# Autodesk Inventor assembly: Monitor
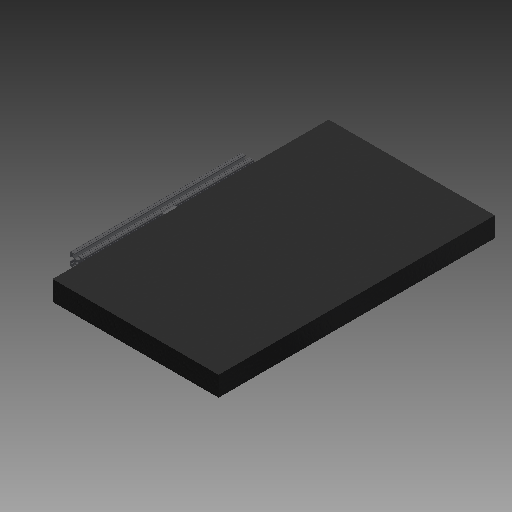
[picture p0: Inventor's stored thumbnail of the model, 512x512]
Saved by Autodesk Inventor 2017 SP1 (Build 210196100, 196)
## iProperties
Created: 2016-04-03
Part Number: Monitor
Document SubType Name: Assembly
Designer: hwasserb
Author: hwasserb
## Documents named in this file (7)
- C:\Users\Haden\Desktop\Charlie-CAD-Model\Robot Model\Monitor\Monitor.iam
- C:\Users\Haden\Desktop\Charlie-CAD-Model\Robot Model\Monitor\Cross Bar.ipt
- C:\Users\Haden\Desktop\Charlie-CAD-Model\Robot Model\Monitor\Monitor.ipt
- C:\Users\Haden\Desktop\Charlie-CAD-Model\Robot Model\Monitor\Vertical Bar.ipt
- C:\Users\Haden\Desktop\Charlie-CAD-Model\Robot Model\Monitor\Lower VESA Mount.ipt
- C:\Users\Haden\Desktop\Charlie-CAD-Model\Robot Model\Monitor\Upper VESA Mount.ipt
- C:\Users\Haden\Desktop\Charlie-CAD-Model\Robot Model\Monitor\Structural Pivot-8020-4198\Structural Pivot-8020-4198.iam
## Components (7 placed, 6 different names)
1. Cross Bar:1 — Mate:15, Flush:4, Flush:5
2. Monitor:1 — Mate:3, Mate:4, Mate:5, Mate:6, Mate:13, Mate:14
3. Vertical Bar:1 — Mate:3, Mate:7, Mate:8, Mate:9, Mate:10, Flush:2, Flush:3, Mate:11, Mate:16, Flush:6, Mate:17
4. Lower VESA Mount:1 — Mate:4, Mate:5, Mate:6, Mate:7, Mate:8
5. Upper VESA Mount:1 — Mate:9, Flush:3, Mate:12, Mate:13
6. Upper VESA Mount:2 — Mate:10, Flush:2, Mate:11, Mate:12, Mate:14
7. Structural Pivot-8020-4198:1 [sub-assembly] — Mate:15, Flush:4, Flush:5, Mate:16, Flush:6, Mate:17
## Relationships (20: Mate 15, Flush 5)
- Mate:3: Monitor:1 ↔ Vertical Bar:1
- Mate:4: Monitor:1 ↔ Lower VESA Mount:1
- Mate:5: Monitor:1 ↔ Lower VESA Mount:1
- Mate:6: Monitor:1 ↔ Lower VESA Mount:1
- Mate:7: Vertical Bar:1 ↔ Lower VESA Mount:1
- Mate:8: Vertical Bar:1 ↔ Lower VESA Mount:1
- Mate:9: Vertical Bar:1 ↔ Upper VESA Mount:1
- Mate:10: Vertical Bar:1 ↔ Upper VESA Mount:2
- Flush:2: Vertical Bar:1 ↔ Upper VESA Mount:2
- Flush:3: Vertical Bar:1 ↔ Upper VESA Mount:1
- Mate:11: Vertical Bar:1 ↔ Upper VESA Mount:2
- Mate:12: Upper VESA Mount:1 ↔ Upper VESA Mount:2
- Mate:13: Monitor:1 ↔ Upper VESA Mount:1
- Mate:14: Monitor:1 ↔ Upper VESA Mount:2
- Mate:15: Cross Bar:1 ↔ Structural Pivot-8020-4198:1
- Flush:4: Cross Bar:1 ↔ Structural Pivot-8020-4198:1
- Flush:5 (152.4 mm): Cross Bar:1 ↔ Structural Pivot-8020-4198:1
- Mate:16: Vertical Bar:1 ↔ Structural Pivot-8020-4198:1
- Flush:6: Vertical Bar:1 ↔ Structural Pivot-8020-4198:1
- Mate:17 (-50.8 mm): Vertical Bar:1 ↔ Structural Pivot-8020-4198:1
